# Autodesk Inventor assembly: Assembly2
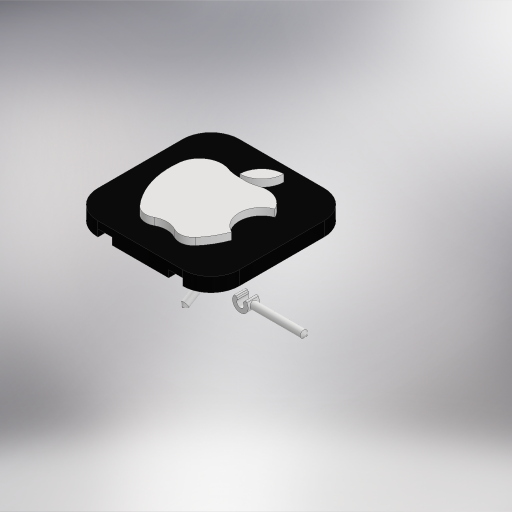
[picture p0: Inventor's stored thumbnail of the model, 512x512]
Saved by Autodesk Inventor 2024 (Build 280153000, 153)
## iProperties
Created: 2023-10-30
Part Number: Assembly2
Document SubType Name: Assembly
Designer: SSAFY
Author: SSAFY
## Documents named in this file (4)
- C:\Users\SSAFY\Desktop\TIL\3D\20231030\Assembly2.iam
- C:\Users\SSAFY\Desktop\TIL\3D\20231030\Apple_logo_Black.ipt
- C:\Users\SSAFY\Desktop\TIL\3D\20231030\Apple_logo_white.ipt
- C:\Users\SSAFY\Desktop\TIL\3D\20231030\Apple_logo_Black_Part2.ipt
## Components (4 placed, 3 different names)
1. Apple_logo_Black:1 — Flush:1, Flush:3, Mate:1, Mate:2, Mate:3
2. Apple_logo_white:1 — Flush:1, Flush:3, Mate:1
3. Apple_logo_Black_Part2:1 — Mate:2, Mate:3
4. Apple_logo_Black_Part2:2
## Relationships (5: Mate 3, Flush 2)
- Flush:1: Apple_logo_Black:1 ↔ Apple_logo_white:1
- Flush:3: Apple_logo_Black:1 ↔ Apple_logo_white:1
- Mate:1: Apple_logo_Black:1 ↔ Apple_logo_white:1
- Mate:2: Apple_logo_Black:1 ↔ Apple_logo_Black_Part2:1
- Mate:3 (2.5 mm): Apple_logo_Black:1 ↔ Apple_logo_Black_Part2:1
